# Autodesk Inventor assembly: Arduino_Mega2560_R3
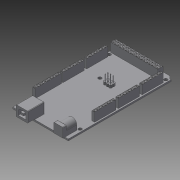
[picture p0: Inventor's stored thumbnail of the model, 180x180]
Saved by Autodesk Inventor 2014 (Build 180170000, 170)
## iProperties
Created: 2014-11-10
Part Number: Arduino_Mega2560_R3
Document SubType Name: Assembly
Designer: ThatOtherGuy
Author: ThatOtherGuy
## Documents named in this file (6)
- C:\Users\ThatOtherGuy\Documents\Inventor\KosselCNC1515\Electronics\Arduino_Mega2560_R3.iam
- C:\Users\ThatOtherGuy\Documents\Inventor\KosselCNC1515\Electronics\Arduino_Mega2560_R3.ipt
- C:\Users\ThatOtherGuy\Documents\Inventor\Content Center Files\R2014\en-US\Header_Female\Header_Female_1x10.ipt
- C:\Users\ThatOtherGuy\Documents\Inventor\Content Center Files\R2014\en-US\Header_Female\Header_Female_1x8.ipt
- C:\Users\ThatOtherGuy\Documents\Inventor\Content Center Files\R2014\en-US\Header_Female\Header_Female_2x18.ipt
- C:\Users\ThatOtherGuy\Documents\Inventor\Content Center Files\R2014\en-US\Header_Male\Header_Male_2x3.ipt
## Components (9 placed, 5 different names)
1. Arduino_Mega2560_R3:1 — Insert:1, Insert:2, Insert:3, Insert:4, Insert:5, Insert:6, Insert:7, Insert:8, Insert:9, Insert:10, Insert:11, Insert:12, Insert:13, Insert:14, Insert:15, Insert:16
2. Header_Female 1-10:1 — Insert:1, Insert:2
3. Header_Female 1-8:1 — Insert:3, Insert:4
4. Header_Female 1-8:2 — Insert:5, Insert:6
5. Header_Female 1-8:3 — Insert:9, Insert:10
6. Header_Female 1-8:4 — Insert:11, Insert:12
7. Header_Female 1-8:5 — Insert:13, Insert:14
8. Header_Female 2-18:1 — Insert:7, Insert:8
9. Header_Male 2-3:1 — Insert:15, Insert:16
## Relationships (16: Insert 16)
- Insert:1: Arduino_Mega2560_R3:1 ↔ Header_Female 1-10:1
- Insert:2: Arduino_Mega2560_R3:1 ↔ Header_Female 1-10:1
- Insert:3: Arduino_Mega2560_R3:1 ↔ Header_Female 1-8:1
- Insert:4: Arduino_Mega2560_R3:1 ↔ Header_Female 1-8:1
- Insert:5: Arduino_Mega2560_R3:1 ↔ Header_Female 1-8:2
- Insert:6: Arduino_Mega2560_R3:1 ↔ Header_Female 1-8:2
- Insert:7: Arduino_Mega2560_R3:1 ↔ Header_Female 2-18:1
- Insert:8: Arduino_Mega2560_R3:1 ↔ Header_Female 2-18:1
- Insert:9: Arduino_Mega2560_R3:1 ↔ Header_Female 1-8:3
- Insert:10: Arduino_Mega2560_R3:1 ↔ Header_Female 1-8:3
- Insert:11: Arduino_Mega2560_R3:1 ↔ Header_Female 1-8:4
- Insert:12: Arduino_Mega2560_R3:1 ↔ Header_Female 1-8:4
- Insert:13: Arduino_Mega2560_R3:1 ↔ Header_Female 1-8:5
- Insert:14: Arduino_Mega2560_R3:1 ↔ Header_Female 1-8:5
- Insert:15: Arduino_Mega2560_R3:1 ↔ Header_Male 2-3:1
- Insert:16: Arduino_Mega2560_R3:1 ↔ Header_Male 2-3:1
